# Autodesk Inventor assembly: Transformador
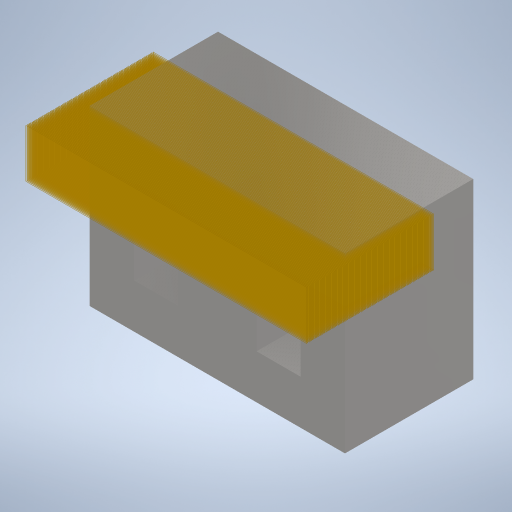
[picture p0: Inventor's stored thumbnail of the model, 512x512]
Saved by Autodesk Inventor 2024.2 (Build 282272000, 272)
## iProperties
Created: 2024-05-06
Part Number: Transformador
Document SubType Name: Assembly
Designer: 082220019
Author: 082220019
## Documents named in this file (3)
- C:\Users\082220019\Downloads\PBL-main\PBL-main\Transformador.iam
- C:\Users\082220019\Downloads\PBL-main\PBL-main\Fechamento.ipt
- C:\Users\082220019\Downloads\PBL-main\PBL-main\Chapa.ipt
## Components (420 placed, 2 different names)
1. Fechamento:1 — Mate:1, Flush:1, Flush:2
2. Chapa:1 — Mate:1, Flush:1, Flush:2
3. Fechamento:2
4. Chapa:2
5. Fechamento:3
6. Chapa:3
7. Fechamento:4
8. Chapa:4
9. Fechamento:5
10. Chapa:5
11. Fechamento:6
12. Chapa:6
13. Fechamento:7
14. Chapa:7
15. Fechamento:8
16. Chapa:8
17. Fechamento:9
18. Chapa:9
19. Fechamento:10
20. Chapa:10
21. Fechamento:11
22. Chapa:11
23. Fechamento:12
24. Chapa:12
25. Fechamento:13
26. Chapa:13
27. Fechamento:14
28. Chapa:14
29. Fechamento:15
30. Chapa:15
31. Fechamento:16
32. Chapa:16
33. Fechamento:17
34. Chapa:17
35. Fechamento:18
36. Chapa:18
37. Fechamento:19
38. Chapa:19
39. Fechamento:20
40. Chapa:20
41. Fechamento:21
42. Chapa:21
43. Fechamento:22
44. Chapa:22
45. Fechamento:23
46. Chapa:23
47. Fechamento:24
48. Chapa:24
49. Fechamento:25
50. Chapa:25
51. Fechamento:26
52. Chapa:26
53. Fechamento:27
54. Chapa:27
55. Fechamento:28
56. Chapa:28
57. Fechamento:29
58. Chapa:29
59. Fechamento:30
60. Chapa:30
61. Fechamento:31
62. Chapa:31
63. Fechamento:32
64. Chapa:32
65. Fechamento:33
66. Chapa:33
67. Fechamento:34
68. Chapa:34
69. Fechamento:35
70. Chapa:35
71. Fechamento:36
72. Chapa:36
73. Fechamento:37
74. Chapa:37
75. Fechamento:38
76. Chapa:38
77. Fechamento:39
78. Chapa:39
79. Fechamento:40
80. Chapa:40
81. Fechamento:41
82. Chapa:41
83. Fechamento:42
84. Chapa:42
85. Fechamento:43
86. Chapa:43
87. Fechamento:44
88. Chapa:44
89. Fechamento:45
90. Chapa:45
91. Fechamento:46
92. Chapa:46
93. Fechamento:47
94. Chapa:47
95. Fechamento:48
96. Chapa:48
97. Fechamento:49
98. Chapa:49
99. Fechamento:50
100. Chapa:50
101. Fechamento:51
102. Chapa:51
103. Fechamento:52
104. Chapa:52
105. Fechamento:53
106. Chapa:53
107. Fechamento:54
108. Chapa:54
109. Fechamento:55
110. Chapa:55
111. Fechamento:56
112. Chapa:56
113. Fechamento:57
114. Chapa:57
115. Fechamento:58
116. Chapa:58
117. Fechamento:59
118. Chapa:59
119. Fechamento:60
120. Chapa:60
121. Fechamento:61
122. Chapa:61
123. Fechamento:62
124. Chapa:62
125. Fechamento:63
126. Chapa:63
127. Fechamento:64
128. Chapa:64
129. Fechamento:65
130. Chapa:65
131. Fechamento:66
132. Chapa:66
133. Fechamento:67
134. Chapa:67
135. Fechamento:68
136. Chapa:68
137. Fechamento:69
138. Chapa:69
139. Fechamento:70
140. Chapa:70
141. Fechamento:71
142. Chapa:71
143. Fechamento:72
144. Chapa:72
145. Fechamento:73
146. Chapa:73
147. Fechamento:74
148. Chapa:74
149. Fechamento:75
150. Chapa:75
151. Fechamento:76
152. Chapa:76
153. Fechamento:77
154. Chapa:77
155. Fechamento:78
156. Chapa:78
157. Fechamento:79
158. Chapa:79
159. Fechamento:80
160. Chapa:80
161. Fechamento:81
162. Chapa:81
163. Fechamento:82
164. Chapa:82
165. Fechamento:83
166. Chapa:83
167. Fechamento:84
168. Chapa:84
169. Fechamento:85
170. Chapa:85
171. Fechamento:86
172. Chapa:86
173. Fechamento:87
174. Chapa:87
175. Fechamento:88
176. Chapa:88
177. Fechamento:89
178. Chapa:89
179. Fechamento:90
180. Chapa:90
181. Fechamento:91
182. Chapa:91
183. Fechamento:92
184. Chapa:92
185. Fechamento:93
186. Chapa:93
187. Fechamento:94
188. Chapa:94
189. Fechamento:95
190. Chapa:95
191. Fechamento:96
192. Chapa:96
193. Fechamento:97
194. Chapa:97
195. Fechamento:98
196. Chapa:98
197. Fechamento:99
198. Chapa:99
199. Fechamento:100
200. Chapa:100
201. Fechamento:101
202. Chapa:101
203. Fechamento:102
204. Chapa:102
205. Fechamento:103
206. Chapa:103
207. Fechamento:104
208. Chapa:104
209. Fechamento:105
210. Chapa:105
211. Fechamento:106
212. Chapa:106
213. Fechamento:107
214. Chapa:107
215. Fechamento:108
216. Chapa:108
217. Fechamento:109
218. Chapa:109
219. Fechamento:110
220. Chapa:110
221. Fechamento:111
222. Chapa:111
223. Fechamento:112
224. Chapa:112
225. Fechamento:113
226. Chapa:113
227. Fechamento:114
228. Chapa:114
229. Fechamento:115
230. Chapa:115
231. Fechamento:116
232. Chapa:116
233. Fechamento:117
234. Chapa:117
235. Fechamento:118
236. Chapa:118
237. Fechamento:119
238. Chapa:119
239. Fechamento:120
240. Chapa:120
241. Fechamento:121
242. Chapa:121
243. Fechamento:122
244. Chapa:122
245. Fechamento:123
246. Chapa:123
247. Fechamento:124
248. Chapa:124
249. Fechamento:125
250. Chapa:125
251. Fechamento:126
252. Chapa:126
253. Fechamento:127
254. Chapa:127
255. Fechamento:128
256. Chapa:128
257. Fechamento:129
258. Chapa:129
259. Fechamento:130
260. Chapa:130
261. Fechamento:131
262. Chapa:131
263. Fechamento:132
264. Chapa:132
265. Fechamento:133
266. Chapa:133
267. Fechamento:134
268. Chapa:134
269. Fechamento:135
270. Chapa:135
271. Fechamento:136
272. Chapa:136
273. Fechamento:137
274. Chapa:137
275. Fechamento:138
276. Chapa:138
277. Fechamento:139
278. Chapa:139
279. Fechamento:140
280. Chapa:140
281. Fechamento:141
282. Chapa:141
283. Fechamento:142
284. Chapa:142
285. Fechamento:143
286. Chapa:143
287. Fechamento:144
288. Chapa:144
289. Fechamento:145
290. Chapa:145
291. Fechamento:146
292. Chapa:146
293. Fechamento:147
294. Chapa:147
295. Fechamento:148
296. Chapa:148
297. Fechamento:149
298. Chapa:149
299. Fechamento:150
300. Chapa:150
301. Fechamento:151
302. Chapa:151
303. Fechamento:152
304. Chapa:152
305. Fechamento:153
306. Chapa:153
307. Fechamento:154
308. Chapa:154
309. Fechamento:155
310. Chapa:155
311. Fechamento:156
312. Chapa:156
313. Fechamento:157
314. Chapa:157
315. Fechamento:158
316. Chapa:158
317. Fechamento:159
318. Chapa:159
319. Fechamento:160
320. Chapa:160
321. Fechamento:161
322. Chapa:161
323. Fechamento:162
324. Chapa:162
325. Fechamento:163
326. Chapa:163
327. Fechamento:164
328. Chapa:164
329. Fechamento:165
330. Chapa:165
331. Fechamento:166
332. Chapa:166
333. Fechamento:167
334. Chapa:167
335. Fechamento:168
336. Chapa:168
337. Fechamento:169
338. Chapa:169
339. Fechamento:170
340. Chapa:170
341. Fechamento:171
342. Chapa:171
343. Fechamento:172
344. Chapa:172
345. Fechamento:173
346. Chapa:173
347. Fechamento:174
348. Chapa:174
349. Fechamento:175
350. Chapa:175
351. Fechamento:176
352. Chapa:176
353. Fechamento:177
354. Chapa:177
355. Fechamento:178
356. Chapa:178
357. Fechamento:179
358. Chapa:179
359. Fechamento:180
360. Chapa:180
361. Fechamento:181
362. Chapa:181
363. Fechamento:182
364. Chapa:182
365. Fechamento:183
366. Chapa:183
367. Fechamento:184
368. Chapa:184
369. Fechamento:185
370. Chapa:185
371. Fechamento:186
372. Chapa:186
373. Fechamento:187
374. Chapa:187
375. Fechamento:188
376. Chapa:188
377. Fechamento:189
378. Chapa:189
379. Fechamento:190
380. Chapa:190
381. Fechamento:191
382. Chapa:191
383. Fechamento:192
384. Chapa:192
385. Fechamento:193
386. Chapa:193
387. Fechamento:194
388. Chapa:194
389. Fechamento:195
390. Chapa:195
391. Fechamento:196
392. Chapa:196
393. Fechamento:197
394. Chapa:197
395. Fechamento:198
396. Chapa:198
397. Fechamento:199
398. Chapa:199
399. Fechamento:200
400. Chapa:200
401. Fechamento:201
402. Chapa:201
403. Fechamento:202
404. Chapa:202
405. Fechamento:203
406. Chapa:203
407. Fechamento:204
408. Chapa:204
409. Fechamento:205
410. Chapa:205
411. Fechamento:206
412. Chapa:206
413. Fechamento:207
414. Chapa:207
415. Fechamento:208
416. Chapa:208
417. Fechamento:209
418. Chapa:209
419. Fechamento:210
420. Chapa:210
## Component patterns: (210 elements, first: Fechamento:1 + Chapa:1)
## Relationships (3: Flush 2, Mate 1)
- Mate:1: Fechamento:1 ↔ Chapa:1
- Flush:1: Fechamento:1 ↔ Chapa:1
- Flush:2: Fechamento:1 ↔ Chapa:1
